# Autodesk Inventor assembly: Top_Assy
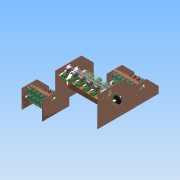
[picture p0: Inventor's stored thumbnail of the model, 180x180]
Saved by Autodesk Inventor 2018.1 (Build 221171000, 171)
## iProperties
Created: 2019-03-18
Part Number: Top_Assy
Document SubType Name: Assembly
Designer: James
Author: James
## Documents named in this file (4)
- C:\Users\admin\Desktop\Ball-Machine\Top Level\Top_Assy.iam
- C:\Users\admin\Desktop\Ball-Machine\Selection Sort\Selection_Assy.iam
- C:\Users\admin\Desktop\Ball-Machine\Pancake Sort\Pancake_Assy.iam
- C:\Users\admin\Desktop\Ball-Machine\Selection Sort\Selection - 4 Lanes\Selection_Assy 4 Lanes.iam
## Components (3 placed, 3 different names)
1. Selection_Assy:1 [sub-assembly] — Flush:1, Flush:2, Flush:3, Flush:4, Flush:5
2. Pancake_Assy:1 [sub-assembly] — Flush:4
3. Selection_Assy 4 Lanes:1 [sub-assembly] — Flush:5
## Relationships (5: Flush 5)
- Flush:1: Selection_Assy:1
- Flush:2: Selection_Assy:1
- Flush:3: Selection_Assy:1
- Flush:4 (110 mm): Selection_Assy:1 ↔ Pancake_Assy:1
- Flush:5: Selection_Assy:1 ↔ Selection_Assy 4 Lanes:1
